# Autodesk Inventor assembly: Enclosure
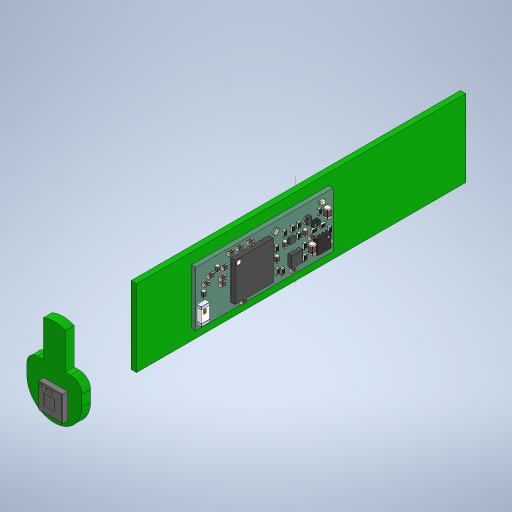
[picture p0: Inventor's stored thumbnail of the model, 512x512]
Saved by Autodesk Inventor 2024 (Build 280153000, 153)
## iProperties
Created: 2025-02-15
Part Number: Enclosure
Document SubType Name: Assembly
Designer: XxPan
Author: XxPan
## Documents named in this file (3)
- C:\Users\XxPan\OneDrive - McMaster University\4OI6\InkSync\case\Enclosure.iam
- C:\Users\XxPan\OneDrive - McMaster University\4OI6\InkSync\case\MCU_PCB.iam
- C:\Users\XxPan\OneDrive - McMaster University\4OI6\InkSync\case\Sensor_PCB.iam
## Components (2 placed, 2 different names)
1. MCU_PCB:1 [sub-assembly] — Angle:1
2. Sensor_PCB:1 [sub-assembly] — Angle:1
## Relationships (1: Angle 1)
- Angle:1 (0 deg): MCU_PCB:1 ↔ Sensor_PCB:1
